# Autodesk Inventor assembly: SchlittenOben
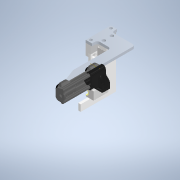
[picture p0: Inventor's stored thumbnail of the model, 180x180]
Saved by Autodesk Inventor 2022 (Build 260153000, 153)
## iProperties
Created: 2022-03-23
Part Number: SchlittenOben
Document SubType Name: Assembly
Designer: kaebi
Author: kaebi
## Documents named in this file (7)
- C:\Users\kaebi\OneDrive - mci4me.at\03_MCI Master\4.Semester_SS2022\Masterarbeit\Software\CAD\106_Vereinzelungseinheit\SchlittenOben.iam
- C:\Users\kaebi\OneDrive - mci4me.at\03_MCI Master\4.Semester_SS2022\Masterarbeit\Software\CAD\106_Vereinzelungseinheit\106.016.01_Schienenfuehrung.ipt
- C:\Users\kaebi\OneDrive - mci4me.at\03_MCI Master\4.Semester_SS2022\Masterarbeit\Software\CAD\106_Vereinzelungseinheit\106.019.01_Distanzplatte.ipt
- C:\Users\kaebi\OneDrive - mci4me.at\03_MCI Master\4.Semester_SS2022\Masterarbeit\Software\CAD\106_Vereinzelungseinheit\106.018.01_Schieberelement_oben.ipt
- C:\Users\kaebi\OneDrive - mci4me.at\03_MCI Master\4.Semester_SS2022\Masterarbeit\Software\CAD\106_Vereinzelungseinheit\106.020.01_Winkelaufnahme_Schwert_unten.ipt
- C:\Users\kaebi\OneDrive - mci4me.at\03_MCI Master\4.Semester_SS2022\Masterarbeit\Software\CAD\106_Vereinzelungseinheit\106.030.01_Schwert_oben.ipt
- C:\Users\kaebi\OneDrive - mci4me.at\03_MCI Master\4.Semester_SS2022\Masterarbeit\Software\CAD\106_Vereinzelungseinheit\206.004.02_Kraftlimitierung.iam
## Components (8 placed, 6 different names)
1. 106.016.01_Schienenfuehrung:1 — Passend:18
2. 106.016.01_Schienenfuehrung:2
3. 106.019.01_Distanzplatte:1
4. 106.018.01_Schieberelement_oben:1 — Passend:18, Passend:19, Passend:20
5. 106.019.01_Distanzplatte:2 — Passend:19, Passend:20
6. 106.020.01_Winkelaufnahme_Schwert_unten:1
7. 106.030.01_Schwert_oben:1
8. 206.004.02_Kraftlimitierung:1 [sub-assembly]
## Relationships (21: Mate 20, Flush 1)
- [Mate]: 106.016.01_Schienenfuehrung:1 ↔ 106.019.01_Distanzplatte:1
- [Mate]: 106.016.01_Schienenfuehrung:2 ↔ 106.019.01_Distanzplatte:2
- [Mate]: 106.019.01_Distanzplatte:1 ↔ 106.018.01_Schieberelement_oben:1
- [Mate]: 106.018.01_Schieberelement_oben:1 ↔ 106.020.01_Winkelaufnahme_Schwert_unten:1
- [Mate]: 106.018.01_Schieberelement_oben:1 ↔ 106.020.01_Winkelaufnahme_Schwert_unten:1
- [Mate]: 106.018.01_Schieberelement_oben:1 ↔ 106.020.01_Winkelaufnahme_Schwert_unten:1
- [Mate]: 106.020.01_Winkelaufnahme_Schwert_unten:1 ↔ 106.030.01_Schwert_oben:1
- [Mate]: 106.018.01_Schieberelement_oben:1 ↔ 206.004.02_Kraftlimitierung:1
- [Mate]: 106.016.01_Schienenfuehrung:2 ↔ 106.019.01_Distanzplatte:2
- [Mate]: 106.016.01_Schienenfuehrung:2 ↔ 106.019.01_Distanzplatte:2
- [Mate]: 106.016.01_Schienenfuehrung:1 ↔ 106.019.01_Distanzplatte:1
- [Mate]: 106.016.01_Schienenfuehrung:1 ↔ 106.019.01_Distanzplatte:1
- [Mate]: 106.019.01_Distanzplatte:1 ↔ 106.018.01_Schieberelement_oben:1
- [Mate]: 106.016.01_Schienenfuehrung:2 ↔ 106.018.01_Schieberelement_oben:1
- [Mate]: 106.018.01_Schieberelement_oben:1 ↔ 206.004.02_Kraftlimitierung:1
- [Mate]: 106.018.01_Schieberelement_oben:1 ↔ 206.004.02_Kraftlimitierung:1
- [Mate]: 106.020.01_Winkelaufnahme_Schwert_unten:1 ↔ 106.030.01_Schwert_oben:1
- [Flush]: 106.020.01_Winkelaufnahme_Schwert_unten:1 ↔ 106.030.01_Schwert_oben:1
- Passend:18 [Mate]: 106.016.01_Schienenfuehrung:1 ↔ 106.018.01_Schieberelement_oben:1
- Passend:19 [Mate]: 106.018.01_Schieberelement_oben:1 ↔ 106.019.01_Distanzplatte:2
- Passend:20 [Mate]: 106.018.01_Schieberelement_oben:1 ↔ 106.019.01_Distanzplatte:2
